# Autodesk Inventor assembly: imu_house_assembly
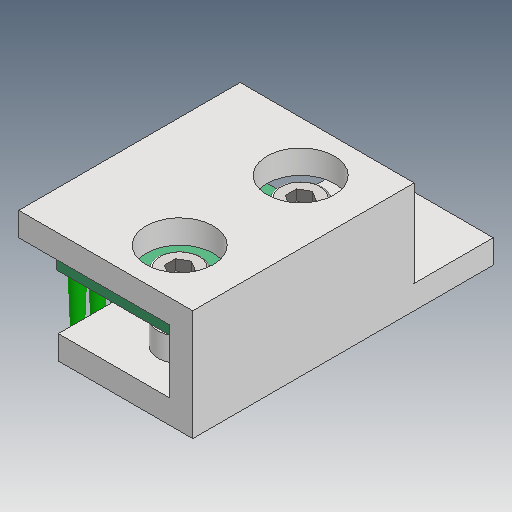
[picture p0: Inventor's stored thumbnail of the model, 512x512]
Saved by Autodesk Inventor 2025.2 (Build 292293000, 293)
## iProperties
Created: 2025-02-13
Part Number: imu_house_assembly
Document SubType Name: Assembly
Designer: Alex
Author: Alex
## Documents named in this file (4)
- C:\Users\email\Desktop\Projects\Capstone\4TB6\CAD_Model\thigh_mount_2\imu_house_assembly.iam
- C:\Users\email\Desktop\Projects\Capstone\4TB6\CAD_Model\thigh_mount_2\IMU_temp.ipt
- C:\Users\email\Desktop\Projects\Capstone\4TB6\CAD_Model\thigh_mount_2\imu_housing_op.ipt
- C:\Users\email\Documents\Inventor\Content Center Files\R2025\en-US\AS 1420\AS 1420 - 1973 - M3 x 6.ipt
## Components (4 placed, 3 different names)
1. IMU_temp:1 — Mate:6, Mate:11, Rigid:1, Rigid:2
2. imu_housing_op:1 — Mate:6, Mate:11
3. AS 1420 - Metric M3 x 6:1 — Rigid:1
4. AS 1420 - Metric M3 x 6:2 — Rigid:2
## Relationships (4: Mate 2, WeldJoint 2)
- Mate:6: IMU_temp:1 ↔ imu_housing_op:1
- Mate:11: IMU_temp:1 ↔ imu_housing_op:1
- Rigid:1 [WeldJoint]: IMU_temp:1 ↔ AS 1420 - Metric M3 x 6:1
- Rigid:2 [WeldJoint]: IMU_temp:1 ↔ AS 1420 - Metric M3 x 6:2
